# Autodesk Inventor assembly: CompleteRobotAssembly_NERDS
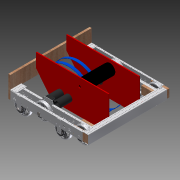
[picture p0: Inventor's stored thumbnail of the model, 180x180]
Saved by Autodesk Inventor 2014 (Build 180170000, 170)
## iProperties
Created: 2016-01-30
Part Number: CompleteRobotAssembly_NERDS
Document SubType Name: Assembly
Designer: bermudezr
Author: bermudezr
## Documents named in this file (3)
- Z:\Nerds_1726\Robot\CompleteRobotAssembly_NERDS.iam
- Z:\Nerds_1726\Robot\Shooting Mechanism\ShooterAssembly_NERDS.iam
- Z:\Nerds_1726\Robot\Chassis\ChassisComplete_NERDS.iam
## Components (2 placed, 2 different names)
1. ShooterAssembly_NERDS:1 [sub-assembly] — Mate:1, Mate:2, Flush:1
2. ChassisComplete_NERDS:1 [sub-assembly] — Mate:1, Mate:2, Flush:1
## Relationships (3: Mate 2, Flush 1)
- Mate:1: ShooterAssembly_NERDS:1 ↔ ChassisComplete_NERDS:1
- Mate:2: ShooterAssembly_NERDS:1 ↔ ChassisComplete_NERDS:1
- Flush:1: ShooterAssembly_NERDS:1 ↔ ChassisComplete_NERDS:1
